# Autodesk Inventor assembly: Main
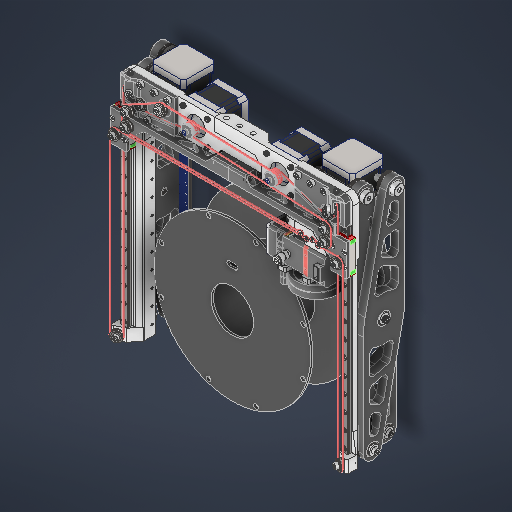
[picture p0: Inventor's stored thumbnail of the model, 512x512]
Saved by Autodesk Inventor 2026.2 (Build 302298000, 298)
## iProperties
Created: 2025-11-20
Part Number: Main
Document SubType Name: Assembly
Designer: gaoet
Author: gaoet
## Documents named in this file (66)
- C:\Users\gaoet\OneDrive\Desktop\Portable3DPrinter\V2\Main.iam
- C:\Users\gaoet\OneDrive\Desktop\Portable3DPrinter\V2\Zeee6S22Ah.ipt
- C:\Users\gaoet\OneDrive\Desktop\Portable3DPrinter\V2\BoundingBox.ipt
- C:\Users\gaoet\OneDrive\Desktop\Portable3DPrinter\V2\BuildVolume.ipt
- C:\Users\gaoet\OneDrive\Desktop\Portable3DPrinter\V2\LaptopScaleModel.ipt
- C:\Users\gaoet\OneDrive\Desktop\Portable3DPrinter\V2\Raspberry PI Zero W\Raspberry PI Zero W.iam
- C:\Users\gaoet\OneDrive\Desktop\Portable3DPrinter\V2\BTT E3 SKR MINI V3.0\BTT E3 SKR MINI V3.0.iam
- C:\Users\gaoet\OneDrive\Desktop\Portable3DPrinter\V2\MGN9-H\MGN9-H\MGN9-H.ipt
- C:\Users\gaoet\OneDrive\Desktop\Portable3DPrinter\V2\ElectronicsBase.ipt
- C:\Users\gaoet\OneDrive\Desktop\Portable3DPrinter\V2\Pololu Stepper with 300mm LeadScrew\Pololu Stepper with 300mm LeadScrew\Pololu Stepper with 300mm LeadScrew.ipt
- C:\Users\gaoet\OneDrive\Desktop\Portable3DPrinter\V2\ScissorArmV2.ipt
- C:\Users\gaoet\OneDrive\Desktop\Portable3DPrinter\V2\7804K117_Stainless Steel Ball Bearing\7804K117_Stainless Steel Ball Bearing\7804K117_Stainless Steel Ball Bearing.ipt
- C:\Users\gaoet\OneDrive\Desktop\Portable3DPrinter\V2\92981A207_Alloy Steel Shoulder Screws\92981A207_Alloy Steel Shoulder Screws\92981A207_Alloy Steel Shoulder Screws.ipt
- C:\Users\gaoet\OneDrive\Desktop\Portable3DPrinter\V2\91415A210_Zinc-Plated Steel Hex Nut\91415A210_Zinc-Plated Steel Hex Nut\91415A210_Zinc-Plated Steel Hex Nut.ipt
- C:\Users\gaoet\OneDrive\Desktop\Portable3DPrinter\V2\CarriagePivotMount.ipt
- C:\Users\gaoet\OneDrive\Desktop\Portable3DPrinter\V2\91290A306_Black-Oxide Alloy Steel Socket Head Screw\91290A306_Black-Oxide Alloy Steel Socket Head Screw\91290A306_Black-Oxide Alloy Steel Socket Head Screw.ipt
- C:\Users\gaoet\OneDrive\Desktop\Portable3DPrinter\V2\PivotWasher.ipt
- C:\Users\gaoet\OneDrive\Desktop\Portable3DPrinter\V2\90591A255_Zinc-Plated Steel Hex Nut\90591A255_Zinc-Plated Steel Hex Nut\90591A255_Zinc-Plated Steel Hex Nut.ipt
- C:\Users\gaoet\OneDrive\Desktop\Portable3DPrinter\V2\ScissorArmV2Inner.ipt
- C:\Users\gaoet\OneDrive\Desktop\Portable3DPrinter\V2\6656K108_Steel Ball Bearing\6656K108_Steel Ball Bearing\6656K108_Steel Ball Bearing.ipt
- C:\Users\gaoet\OneDrive\Desktop\Portable3DPrinter\V2\91290A168_Black-Oxide Alloy Steel Socket Head Screw\91290A168_Black-Oxide Alloy Steel Socket Head Screw\91290A168_Black-Oxide Alloy Steel Socket Head Screw.ipt
- C:\Users\gaoet\OneDrive\Desktop\Portable3DPrinter\V2\ThrustBearing.iam
- C:\Users\gaoet\OneDrive\Desktop\Portable3DPrinter\V2\MGN9-C v2 v0\MGN9-C v2.iam
- C:\Users\gaoet\OneDrive\Desktop\Portable3DPrinter\V2\UpperCarriagePivotMount.ipt
- C:\Users\gaoet\OneDrive\Desktop\Portable3DPrinter\V2\MGN9-H\MGN9-H\MGN9-H_MIR.ipt
- C:\Users\gaoet\OneDrive\Desktop\Portable3DPrinter\V2\91415A210_Zinc-Plated Steel Hex Nut\91415A210_Zinc-Plated Steel Hex Nut\91415A210_Zinc-Plated Steel Hex Nut_MIR.ipt
- C:\Users\gaoet\OneDrive\Desktop\Portable3DPrinter\V2\7804K117_Stainless Steel Ball Bearing\7804K117_Stainless Steel Ball Bearing\7804K117_Stainless Steel Ball Bearing_MIR.ipt
- C:\Users\gaoet\OneDrive\Desktop\Portable3DPrinter\V2\ScissorArmV2_MIR.ipt
- C:\Users\gaoet\OneDrive\Desktop\Portable3DPrinter\V2\92981A207_Alloy Steel Shoulder Screws\92981A207_Alloy Steel Shoulder Screws\92981A207_Alloy Steel Shoulder Screws_MIR.ipt
- C:\Users\gaoet\OneDrive\Desktop\Portable3DPrinter\V2\CarriagePivotMount_MIR.ipt
- C:\Users\gaoet\OneDrive\Desktop\Portable3DPrinter\V2\91290A306_Black-Oxide Alloy Steel Socket Head Screw\91290A306_Black-Oxide Alloy Steel Socket Head Screw\91290A306_Black-Oxide Alloy Steel Socket Head Screw_MIR.ipt
- C:\Users\gaoet\OneDrive\Desktop\Portable3DPrinter\V2\PivotWasher_MIR.ipt
- C:\Users\gaoet\OneDrive\Desktop\Portable3DPrinter\V2\90591A255_Zinc-Plated Steel Hex Nut\90591A255_Zinc-Plated Steel Hex Nut\90591A255_Zinc-Plated Steel Hex Nut_MIR.ipt
- C:\Users\gaoet\OneDrive\Desktop\Portable3DPrinter\V2\ScissorArmV2Inner_MIR.ipt
- C:\Users\gaoet\OneDrive\Desktop\Portable3DPrinter\V2\6656K108_Steel Ball Bearing\6656K108_Steel Ball Bearing\6656K108_Steel Ball Bearing_MIR.ipt
- C:\Users\gaoet\OneDrive\Desktop\Portable3DPrinter\V2\91290A168_Black-Oxide Alloy Steel Socket Head Screw\91290A168_Black-Oxide Alloy Steel Socket Head Screw\91290A168_Black-Oxide Alloy Steel Socket Head Screw_MIR.ipt
- C:\Users\gaoet\OneDrive\Desktop\Portable3DPrinter\V2\ThrustBearing_MIR.iam
- C:\Users\gaoet\OneDrive\Desktop\Portable3DPrinter\V2\MGN9-C v2 v0\MGN9-C v2_MIR.iam
- C:\Users\gaoet\OneDrive\Desktop\Portable3DPrinter\V2\UpperCarriagePivotMount_MIR.ipt
- C:\Users\gaoet\OneDrive\Desktop\Portable3DPrinter\V2\91290A110_Black-Oxide Alloy Steel Socket Head Screw\91290A110_Black-Oxide Alloy Steel Socket Head Screw\91290A110_Black-Oxide Alloy Steel Socket Head Screw_MIR.ipt
- C:\Users\gaoet\OneDrive\Desktop\Portable3DPrinter\V2\GantryRailMount_MIR.ipt
- C:\Users\gaoet\OneDrive\Desktop\Portable3DPrinter\V2\Extruder.iam
- C:\Users\gaoet\OneDrive\Desktop\Portable3DPrinter\V2\MGNRail250mm.ipt
- C:\Users\gaoet\OneDrive\Desktop\Portable3DPrinter\V2\XGantryMount.ipt
- C:\Users\gaoet\OneDrive\Desktop\Portable3DPrinter\V2\BearingU604.ipt
- C:\Users\gaoet\OneDrive\Desktop\Portable3DPrinter\V2\90729A168_Passivated 316 Stainless Steel Hex-Drive Flat Head Screw\90729A168_Passivated 316 Stainless Steel Hex-Drive Flat Head Screw\90729A168_Passivated 316 .ipt
- C:\Users\gaoet\OneDrive\Desktop\Portable3DPrinter\V2\ElevatorPlate.ipt
- C:\Users\gaoet\OneDrive\Desktop\Portable3DPrinter\V2\ElevatorPlate_MIR.ipt
- C:\Users\gaoet\OneDrive\Desktop\Portable3DPrinter\V2\XGantryMount_MIR.ipt
- C:\Users\gaoet\OneDrive\Desktop\Portable3DPrinter\V2\Pulley.ipt
- C:\Users\gaoet\OneDrive\Desktop\Portable3DPrinter\V2\Tensioner.ipt
- C:\Users\gaoet\OneDrive\Desktop\Portable3DPrinter\V2\PSU.ipt
- C:\Users\gaoet\OneDrive\Desktop\Portable3DPrinter\V2\FrontPanel.ipt
- C:\Users\gaoet\OneDrive\Desktop\Portable3DPrinter\V2\BTT Mini 12864 V1.0\BTT Mini 12864 V1.0\BTT Mini 12864 V1.0.ipt
- C:\Users\gaoet\OneDrive\Desktop\Portable3DPrinter\V2\RightTruss.ipt
- C:\Users\gaoet\OneDrive\Desktop\Portable3DPrinter\V2\LeftTruss.ipt
- C:\Users\gaoet\OneDrive\Desktop\Portable3DPrinter\V2\RoutingPlateV2.ipt
- C:\Users\gaoet\OneDrive\Desktop\Portable3DPrinter\V2\RoutingPlateV2Right.ipt
- C:\Users\gaoet\OneDrive\Desktop\Portable3DPrinter\V2\92095A181_NO THREADS_18-8 Stainless Steel Button Head Hex-Drive Screw\92095A181_NO THREADS_18-8 Stainless Steel Button Head Hex-Drive Screw\92095A181_NO THREAD.ipt
- C:\Users\gaoet\OneDrive\Desktop\Portable3DPrinter\V2\MockCable.ipt
- C:\Users\gaoet\OneDrive\Desktop\Portable3DPrinter\V2\MockCable2.ipt
- C:\Users\gaoet\OneDrive\Desktop\Portable3DPrinter\V2\Banana\Banana\Banana.ipt
- C:\Users\gaoet\OneDrive\Desktop\Portable3DPrinter\V2\GantryRailMount.ipt
- C:\Users\gaoet\OneDrive\Desktop\Portable3DPrinter\V2\cardboard spool v1\cardboard spool v1\cardboard spool v1.ipt
- C:\Users\gaoet\OneDrive\Desktop\Portable3DPrinter\Scissor 3D Printer\Nema17x38mm.ipt
- C:\Users\gaoet\OneDrive\Desktop\Portable3DPrinter\Scissor 3D Printer\Pololu Stepper with 300mm LeadScrew\Pololu Stepper with 300mm LeadScrew\Pololu Stepper with 300mm LeadScrew.ipt
## Components (259 placed, 64 different names)
1. Zeee6S22Ah:1
2. BoundingBox:1 — Angle:2, Mate:149, Flush:47
3. BuildVolume:1
4. LaptopScaleModel:1
5. Raspberry PI Zero W:1 [sub-assembly] — Insert:264, Insert:265
6. BTT E3 SKR MINI V3.0:1 [sub-assembly]
7. MGN9-H:2 — Insert:39, Mate:61, Mate:185
8. MGN9-H:3 — Mate:111, Flush:33, Insert:310
9. MGN9-H:6 — Mate:112, Flush:30, Insert:123, Mate:116
10. ElectronicsBase:1 — Mate:149, Flush:47, Mate:156, Flush:49, Insert:203, Insert:206, Insert:210, Insert:214, Insert:215
11. 91415A210_Zinc-Plated Steel Hex Nut:1 — Mate:56
12. 7804K117_Stainless Steel Ball Bearing:2 — Mate:70, Insert:52, Insert:325
13. ScissorArmV2:3 — Insert:35, Angle:2, Mate:73, Insert:63, Insert:64, Insert:71, Insert:74, Insert:78, Angle:4
14. 7804K117_Stainless Steel Ball Bearing:3 — Insert:35, Insert:37
15. 92981A207_Alloy Steel Shoulder Screws:3 — Insert:37, Mate:56
16. CarriagePivotMount:1 — Insert:39, Mate:61, Insert:53, Insert:72
17. 91290A306_Black-Oxide Alloy Steel Socket Head Screw:1 — Mate:70, Insert:51
18. PivotWasher:1 — Insert:51, Insert:52
19. 90591A255_Zinc-Plated Steel Hex Nut:1 — Insert:53
20. ScissorArmV2Inner:1 — Mate:73, Insert:68, Mate:74, Insert:73, Angle:4, Insert:316, Insert:325, Insert:326
21. 7804K117_Stainless Steel Ball Bearing:6 — Insert:63, Insert:66
22. 6656K108_Steel Ball Bearing:1 — Insert:64, Insert:65
23. 6656K108_Steel Ball Bearing:2 — Insert:65
24. PivotWasher:3 — Insert:66, Insert:67
25. 91290A168_Black-Oxide Alloy Steel Socket Head Screw:2 — Insert:67
26. 90591A255_Zinc-Plated Steel Hex Nut:2 — Insert:68, Mate:74
27. ThrustBearing:1 [sub-assembly] — Insert:71
28. ThrustBearing:2 [sub-assembly] — Insert:72, Insert:73
29. MGN9-C v2:1 [sub-assembly] — Mate:80, Insert:308, Flush:51
30. 7804K117_Stainless Steel Ball Bearing:7 — Insert:74, Insert:76
31. PivotWasher:4 — Insert:76, Insert:88
32. ThrustBearing:3 [sub-assembly] — Insert:78, Mate:77, Mate:78
33. UpperCarriagePivotMount:1 — Mate:77, Mate:78, Mate:80, Insert:89, Mate:89, Insert:292, Insert:293, Insert:294, Insert:295, Insert:308
34. 91290A306_Black-Oxide Alloy Steel Socket Head Screw:3 — Insert:88
35. 90591A255_Zinc-Plated Steel Hex Nut:3 — Insert:89, Mate:89
36. MGN9-H_MIR:1 — Mate:94, Insert:93
37. 91415A210_Zinc-Plated Steel Hex Nut_MIR:1 — Mate:93
38. 7804K117_Stainless Steel Ball Bearing_MIR:1 — Mate:95, Insert:94, Insert:324
39. ScissorArmV2_MIR:1 — Insert:90, Angle:6, Mate:96, Insert:98, Insert:99, Insert:104, Insert:107, Insert:109
40. 7804K117_Stainless Steel Ball Bearing_MIR:2 — Insert:90, Insert:91
41. 92981A207_Alloy Steel Shoulder Screws_MIR:1 — Mate:93, Insert:91
42. CarriagePivotMount_MIR:1 — Mate:94, Insert:93, Insert:96, Insert:106
43. 91290A306_Black-Oxide Alloy Steel Socket Head Screw_MIR:1 — Mate:95, Insert:95
44. PivotWasher_MIR:1 — Insert:94, Insert:95
45. 90591A255_Zinc-Plated Steel Hex Nut_MIR:1 — Insert:96
46. ScissorArmV2Inner_MIR:1 — Angle:6, Mate:96, Mate:97, Insert:103, Insert:105, Insert:317, Insert:324, Insert:327, Mate:186
47. 7804K117_Stainless Steel Ball Bearing_MIR:3 — Insert:98, Insert:101
48. 6656K108_Steel Ball Bearing_MIR:1 — Insert:99, Insert:100
49. 6656K108_Steel Ball Bearing_MIR:2 — Insert:100, Mate:186
50. PivotWasher_MIR:2 — Insert:101, Insert:102
51. 91290A168_Black-Oxide Alloy Steel Socket Head Screw_MIR:1 — Insert:102
52. 90591A255_Zinc-Plated Steel Hex Nut_MIR:2 — Mate:97, Insert:103
53. ThrustBearing_MIR:1 [sub-assembly] — Insert:104
54. ThrustBearing_MIR:2 [sub-assembly] — Insert:105, Insert:106
55. MGN9-C v2_MIR:1 [sub-assembly] — Mate:99, Mate:122, Flush:35, Insert:307
56. 7804K117_Stainless Steel Ball Bearing_MIR:4 — Insert:107, Insert:108
57. PivotWasher_MIR:3 — Insert:108, Insert:116
58. ThrustBearing_MIR:3 [sub-assembly] — Insert:109, Mate:100, Mate:101
59. UpperCarriagePivotMount_MIR:1 — Mate:99, Mate:100, Mate:101, Mate:106, Insert:117, Insert:296, Insert:297, Insert:298, Insert:299, Insert:307
60. 91290A306_Black-Oxide Alloy Steel Socket Head Screw_MIR:2 — Insert:116
61. 90591A255_Zinc-Plated Steel Hex Nut_MIR:3 — Mate:106, Insert:117
62. Extruder:1 [sub-assembly] — Insert:310, Insert:311, Insert:312, Insert:313, Insert:314
63. MGNRail250mm:3 — Mate:111, Insert:124, Flush:33, Mate:117, Insert:260
64. MGNRail250mm:4 — Mate:112, Flush:30, Insert:152, Mate:128, Insert:319, Insert:320
65. XGantryMount:1 — Insert:123, Mate:116, Insert:124, Mate:117, Insert:138, Insert:139, Insert:140, Insert:141, Mate:126, Insert:142, Insert:145, Mate:131, Flush:42, Insert:183, Insert:184, Mate:174, Angle:12
66. GantryRailMount_MIR:1 — Insert:132, Insert:133, Insert:134, Insert:135, Insert:153
67. MGNRail250mm:6 — Mate:122, Flush:35, Insert:132, Insert:133, Insert:287
68. MGN9-H:7 — Insert:154, Mate:135
69. MGNRail250mm:7 — Insert:134, Insert:135, Insert:247, Mate:188
70. BearingU604:1 — Insert:147, Insert:321
71. BearingU604:2 — Insert:145, Insert:146
72. BearingU604:3 — Mate:126, Insert:142, Insert:143
73. BearingU604:4 — Insert:156, Insert:158, Mate:178
74. BearingU604:5 — Insert:155, Insert:159
75. BearingU604:6 — Insert:153, Insert:157, Mate:179
76. 90729A168_Passivated 316 :1 — Insert:140
77. 90729A168_Passivated 316 :2 — Insert:141
78. 90729A168_Passivated 316 :3 — Insert:139
79. 90729A168_Passivated 316 :4 — Insert:138
80. 91290A306_Black-Oxide Alloy Steel Socket Head Screw:4 — Insert:143, Mate:175
81. 91290A306_Black-Oxide Alloy Steel Socket Head Screw:5 — Insert:146
82. 91290A306_Black-Oxide Alloy Steel Socket Head Screw:6 — Insert:147
83. 90729A168_Passivated 316 :5 — Insert:312
84. 90729A168_Passivated 316 :6 — Insert:313
85. 90729A168_Passivated 316 :7 — Mate:173, Insert:314
86. 90729A168_Passivated 316 :8 — Insert:311
87. ElevatorPlate:1 — Insert:152, Mate:128, Mate:131, Flush:40, Flush:41, Insert:216, Insert:217, Insert:258, Mate:180, Insert:322, Insert:323, Insert:334, Mate:189
88. ElevatorPlate_MIR:1 — Flush:40, Flush:41, Insert:223, Insert:259, Mate:180, Mate:188, Insert:335, Mate:190
89. XGantryMount_MIR:1 — Insert:154, Mate:135, Flush:42, Insert:155, Insert:156, Insert:160, Insert:161, Insert:162, Insert:163
90. 91290A306_Black-Oxide Alloy Steel Socket Head Screw:7 — Insert:157
91. 91290A306_Black-Oxide Alloy Steel Socket Head Screw:8 — Insert:158
92. 91290A306_Black-Oxide Alloy Steel Socket Head Screw:9 — Insert:159
93. 90729A168_Passivated 316 :9 — Insert:163
94. 90729A168_Passivated 316 :10 — Insert:162
95. 90729A168_Passivated 316 :11 — Insert:161
96. 90729A168_Passivated 316 :12 — Insert:160
97. 92981A207_Alloy Steel Shoulder Screws:4 — Insert:165
98. ThrustBearing:4 [sub-assembly] — Insert:316
99. 7804K117_Stainless Steel Ball Bearing:8 — Insert:165, Insert:326
100. 91415A210_Zinc-Plated Steel Hex Nut:3
101. 92981A207_Alloy Steel Shoulder Screws:5 — Insert:176
102. ThrustBearing:5 [sub-assembly] — Insert:317
103. 7804K117_Stainless Steel Ball Bearing_MIR:5 — Insert:176, Insert:327
104. MGNRail250mm:8 — Mate:185
105. MGNRail250mm:9 — Insert:285
106. BearingU604:10 — Insert:218, Insert:219
107. BearingU604:12 — Insert:187
108. 91290A306_Black-Oxide Alloy Steel Socket Head Screw:20 — Insert:184
109. 91290A306_Black-Oxide Alloy Steel Socket Head Screw:21 — Insert:183
110. Pulley:1 — Mate:192, Flush:55
111. Pulley:2 — Mate:191, Flush:55
112. BearingU604:17 — Insert:229, Insert:231
113. Tensioner:1 — Insert:187, Mate:159, Insert:220, Mate:176, Mate:182
114. PSU:1
115. FrontPanel:2 — Mate:156, Flush:49, Angle:11, Insert:199, Insert:200
116. BTT Mini 12864 V1.0:1 — Angle:11, Insert:199, Insert:200
117. 90729A168_Passivated 316 :15 — Insert:203
118. 90729A168_Passivated 316 :16 — Insert:206
119. 90729A168_Passivated 316 :17 — Insert:210
120. RightTruss:1
121. LeftTruss:1
122. 90729A168_Passivated 316 :19 — Insert:214
123. 90729A168_Passivated 316 :20 — Insert:215
124. RoutingPlateV2:1 — Insert:216, Insert:217, Mate:159, Insert:218, Insert:221, Insert:248, Insert:249, Insert:250, Insert:251, Insert:257, Mate:176, Mate:182
125. 91290A306_Black-Oxide Alloy Steel Socket Head Screw:22 — Insert:219
126. 91290A306_Black-Oxide Alloy Steel Socket Head Screw:23 — Insert:220
127. BearingU604:18 — Insert:221, Insert:222
128. 91290A306_Black-Oxide Alloy Steel Socket Head Screw:24 — Insert:222
129. RoutingPlateV2Right:1 — Insert:223, Insert:225, Mate:164, Insert:228, Insert:229, Insert:252, Insert:253, Insert:254, Insert:255, Insert:256, Mate:177, Mate:183
130. BearingU604:19 — Insert:225, Insert:232
131. BearingU604:21
132. Tensioner:2 — Mate:164, Mate:177, Mate:183
133. 91290A306_Black-Oxide Alloy Steel Socket Head Screw:25
134. BearingU604:22 — Insert:228, Insert:230
135. 91290A306_Black-Oxide Alloy Steel Socket Head Screw:26 — Insert:230
136. 91290A306_Black-Oxide Alloy Steel Socket Head Screw:27 — Insert:231
137. 91290A306_Black-Oxide Alloy Steel Socket Head Screw:28 — Insert:232
138. 91290A306_Black-Oxide Alloy Steel Socket Head Screw:29 — Insert:249
139. 91290A306_Black-Oxide Alloy Steel Socket Head Screw:30 — Insert:251
140. 91290A306_Black-Oxide Alloy Steel Socket Head Screw:31 — Insert:250
141. 91290A306_Black-Oxide Alloy Steel Socket Head Screw:32 — Insert:248
142. 91290A306_Black-Oxide Alloy Steel Socket Head Screw:33 — Insert:255
143. 91290A306_Black-Oxide Alloy Steel Socket Head Screw:34 — Insert:254
144. 91290A306_Black-Oxide Alloy Steel Socket Head Screw:35 — Insert:252
145. 91290A306_Black-Oxide Alloy Steel Socket Head Screw:36 — Insert:253
146. 91290A110_Black-Oxide Alloy Steel Socket Head Screw_MIR:31 — Insert:257
147. 91290A110_Black-Oxide Alloy Steel Socket Head Screw_MIR:32 — Insert:256
148. 91290A110_Black-Oxide Alloy Steel Socket Head Screw_MIR:61 — Insert:264
149. 91290A110_Black-Oxide Alloy Steel Socket Head Screw_MIR:62 — Insert:265
150. 91290A306_Black-Oxide Alloy Steel Socket Head Screw:55
151. 91290A110_Black-Oxide Alloy Steel Socket Head Screw_MIR:115
152. 91290A110_Black-Oxide Alloy Steel Socket Head Screw_MIR:116
153. 91290A110_Black-Oxide Alloy Steel Socket Head Screw_MIR:117
154. 91290A110_Black-Oxide Alloy Steel Socket Head Screw_MIR:118
155. 92095A181_NO THREAD:1 — Insert:295
156. 92095A181_NO THREAD:2 — Insert:294
157. 92095A181_NO THREAD:3 — Insert:293
158. 92095A181_NO THREAD:4 — Insert:292
159. 92095A181_NO THREAD:5 — Insert:296
160. 92095A181_NO THREAD:6 — Insert:297
161. 92095A181_NO THREAD:7 — Insert:298
162. 92095A181_NO THREAD:8 — Insert:299
163. MockCable:1 — Mate:173, Mate:174, Angle:12, Mate:175
164. MockCable2:1 — Mate:178, Mate:179
165. Banana:1
166. GantryRailMount:1 — Insert:319, Insert:320, Insert:321
167. MGNRail250mm:10 — Insert:322, Insert:323, Flush:51
168. cardboard spool v1:1
169. Pololu Stepper with 300mm LeadScrew:2
170. Nema17x38mm:1 — Insert:334, Mate:189, Mate:192
171. Nema17x38mm:2 — Insert:335, Mate:190, Mate:191
172. Pololu Stepper with 300mm LeadScrew:3
173. Pololu Stepper with 300mm LeadScrew:4
174. 91290A110_Black-Oxide Alloy Steel Socket Head Screw_MIR:5 — Insert:247
175. 91290A110_Black-Oxide Alloy Steel Socket Head Screw_MIR:18
176. 91290A110_Black-Oxide Alloy Steel Socket Head Screw_MIR:6
177. 91290A110_Black-Oxide Alloy Steel Socket Head Screw_MIR:19
178. 91290A110_Black-Oxide Alloy Steel Socket Head Screw_MIR:7
179. 91290A110_Black-Oxide Alloy Steel Socket Head Screw_MIR:20
180. 91290A110_Black-Oxide Alloy Steel Socket Head Screw_MIR:8
181. 91290A110_Black-Oxide Alloy Steel Socket Head Screw_MIR:21
182. 91290A110_Black-Oxide Alloy Steel Socket Head Screw_MIR:9
183. 91290A110_Black-Oxide Alloy Steel Socket Head Screw_MIR:22
184. 91290A110_Black-Oxide Alloy Steel Socket Head Screw_MIR:10
185. 91290A110_Black-Oxide Alloy Steel Socket Head Screw_MIR:23
186. 91290A110_Black-Oxide Alloy Steel Socket Head Screw_MIR:11
187. 91290A110_Black-Oxide Alloy Steel Socket Head Screw_MIR:24
188. 91290A110_Black-Oxide Alloy Steel Socket Head Screw_MIR:12
189. 91290A110_Black-Oxide Alloy Steel Socket Head Screw_MIR:25
190. 91290A110_Black-Oxide Alloy Steel Socket Head Screw_MIR:13
191. 91290A110_Black-Oxide Alloy Steel Socket Head Screw_MIR:26
192. 91290A110_Black-Oxide Alloy Steel Socket Head Screw_MIR:14
193. 91290A110_Black-Oxide Alloy Steel Socket Head Screw_MIR:27
194. 91290A110_Black-Oxide Alloy Steel Socket Head Screw_MIR:15
195. 91290A110_Black-Oxide Alloy Steel Socket Head Screw_MIR:28
196. 91290A110_Black-Oxide Alloy Steel Socket Head Screw_MIR:16
197. 91290A110_Black-Oxide Alloy Steel Socket Head Screw_MIR:29
198. 91290A110_Black-Oxide Alloy Steel Socket Head Screw_MIR:17
199. 91290A110_Black-Oxide Alloy Steel Socket Head Screw_MIR:30
200. 91290A110_Black-Oxide Alloy Steel Socket Head Screw_MIR:41 — Insert:260
201. 91290A110_Black-Oxide Alloy Steel Socket Head Screw_MIR:42
202. 91290A110_Black-Oxide Alloy Steel Socket Head Screw_MIR:43
203. 91290A110_Black-Oxide Alloy Steel Socket Head Screw_MIR:44
204. 91290A110_Black-Oxide Alloy Steel Socket Head Screw_MIR:45
205. 91290A110_Black-Oxide Alloy Steel Socket Head Screw_MIR:46
206. 91290A110_Black-Oxide Alloy Steel Socket Head Screw_MIR:47
207. 91290A110_Black-Oxide Alloy Steel Socket Head Screw_MIR:48
208. 91290A110_Black-Oxide Alloy Steel Socket Head Screw_MIR:49
209. 91290A110_Black-Oxide Alloy Steel Socket Head Screw_MIR:50
210. 91290A110_Black-Oxide Alloy Steel Socket Head Screw_MIR:51
211. 91290A110_Black-Oxide Alloy Steel Socket Head Screw_MIR:52
212. 91290A110_Black-Oxide Alloy Steel Socket Head Screw_MIR:53
213. 91290A110_Black-Oxide Alloy Steel Socket Head Screw_MIR:63 — Insert:285
214. 91290A110_Black-Oxide Alloy Steel Socket Head Screw_MIR:64
215. 91290A110_Black-Oxide Alloy Steel Socket Head Screw_MIR:65
216. 91290A110_Black-Oxide Alloy Steel Socket Head Screw_MIR:66
217. 91290A110_Black-Oxide Alloy Steel Socket Head Screw_MIR:67
218. 91290A110_Black-Oxide Alloy Steel Socket Head Screw_MIR:68
219. 91290A110_Black-Oxide Alloy Steel Socket Head Screw_MIR:69
220. 91290A110_Black-Oxide Alloy Steel Socket Head Screw_MIR:70
221. 91290A110_Black-Oxide Alloy Steel Socket Head Screw_MIR:71
222. 91290A110_Black-Oxide Alloy Steel Socket Head Screw_MIR:72
223. 91290A110_Black-Oxide Alloy Steel Socket Head Screw_MIR:73
224. 91290A110_Black-Oxide Alloy Steel Socket Head Screw_MIR:74
225. 91290A110_Black-Oxide Alloy Steel Socket Head Screw_MIR:75
226. 91290A110_Black-Oxide Alloy Steel Socket Head Screw_MIR:76
227. 91290A110_Black-Oxide Alloy Steel Socket Head Screw_MIR:77
228. 91290A110_Black-Oxide Alloy Steel Socket Head Screw_MIR:78
229. 91290A110_Black-Oxide Alloy Steel Socket Head Screw_MIR:79
230. 91290A110_Black-Oxide Alloy Steel Socket Head Screw_MIR:80
231. 91290A110_Black-Oxide Alloy Steel Socket Head Screw_MIR:81
232. 91290A110_Black-Oxide Alloy Steel Socket Head Screw_MIR:82
233. 91290A110_Black-Oxide Alloy Steel Socket Head Screw_MIR:83
234. 91290A110_Black-Oxide Alloy Steel Socket Head Screw_MIR:84
235. 91290A110_Black-Oxide Alloy Steel Socket Head Screw_MIR:85
236. 91290A110_Black-Oxide Alloy Steel Socket Head Screw_MIR:86
237. 91290A110_Black-Oxide Alloy Steel Socket Head Screw_MIR:87
238. 91290A110_Black-Oxide Alloy Steel Socket Head Screw_MIR:88
239. 91290A110_Black-Oxide Alloy Steel Socket Head Screw_MIR:102 — Insert:287
240. 91290A110_Black-Oxide Alloy Steel Socket Head Screw_MIR:103
241. 91290A110_Black-Oxide Alloy Steel Socket Head Screw_MIR:104
242. 91290A110_Black-Oxide Alloy Steel Socket Head Screw_MIR:105
243. 91290A110_Black-Oxide Alloy Steel Socket Head Screw_MIR:106
244. 91290A110_Black-Oxide Alloy Steel Socket Head Screw_MIR:107
245. 91290A110_Black-Oxide Alloy Steel Socket Head Screw_MIR:108
246. 91290A110_Black-Oxide Alloy Steel Socket Head Screw_MIR:109
247. 91290A110_Black-Oxide Alloy Steel Socket Head Screw_MIR:110
248. 91290A110_Black-Oxide Alloy Steel Socket Head Screw_MIR:111
249. 91290A110_Black-Oxide Alloy Steel Socket Head Screw_MIR:112
250. 91290A110_Black-Oxide Alloy Steel Socket Head Screw_MIR:113
251. 91290A110_Black-Oxide Alloy Steel Socket Head Screw_MIR:114
252. 91290A110_Black-Oxide Alloy Steel Socket Head Screw_MIR:33 — Insert:258
253. 91290A110_Black-Oxide Alloy Steel Socket Head Screw_MIR:130
254. 91290A110_Black-Oxide Alloy Steel Socket Head Screw_MIR:131
255. 91290A110_Black-Oxide Alloy Steel Socket Head Screw_MIR:132
256. 91290A110_Black-Oxide Alloy Steel Socket Head Screw_MIR:37 — Insert:259
257. 91290A110_Black-Oxide Alloy Steel Socket Head Screw_MIR:133
258. 91290A110_Black-Oxide Alloy Steel Socket Head Screw_MIR:134
259. 91290A110_Black-Oxide Alloy Steel Socket Head Screw_MIR:135
## Component patterns: (26 elements, first: 91290A110_Black-Oxide Alloy Steel Socket Head Screw_MIR:5), (13 elements, first: 91290A110_Black-Oxide Alloy Steel Socket Head Screw_MIR:41), (26 elements, first: 91290A110_Black-Oxide Alloy Steel Socket Head Screw_MIR:63), (13 elements, first: 91290A110_Black-Oxide Alloy Steel Socket Head Screw_MIR:102), (4 elements, first: 91290A110_Black-Oxide Alloy Steel Socket Head Screw_MIR:33), (4 elements, first: 91290A110_Black-Oxide Alloy Steel Socket Head Screw_MIR:37)
## Relationships (206: Insert 141, Mate 49, Flush 11, Angle 5)
- Insert:35: ScissorArmV2:3 ↔ 7804K117_Stainless Steel Ball Bearing:3
- Insert:37: 7804K117_Stainless Steel Ball Bearing:3 ↔ 92981A207_Alloy Steel Shoulder Screws:3
- Mate:56: 91415A210_Zinc-Plated Steel Hex Nut:1 ↔ 92981A207_Alloy Steel Shoulder Screws:3
- Angle:2 (186 deg): BoundingBox:1 ↔ ScissorArmV2:3
- Insert:39: MGN9-H:2 ↔ CarriagePivotMount:1
- Mate:61: MGN9-H:2 ↔ CarriagePivotMount:1
- Mate:70: 7804K117_Stainless Steel Ball Bearing:2 ↔ 91290A306_Black-Oxide Alloy Steel Socket Head Screw:1
- Insert:51: 91290A306_Black-Oxide Alloy Steel Socket Head Screw:1 ↔ PivotWasher:1
- Insert:52: 7804K117_Stainless Steel Ball Bearing:2 ↔ PivotWasher:1
- Insert:53: CarriagePivotMount:1 ↔ 90591A255_Zinc-Plated Steel Hex Nut:1
- Mate:73: ScissorArmV2:3 ↔ ScissorArmV2Inner:1
- Insert:63: ScissorArmV2:3 ↔ 7804K117_Stainless Steel Ball Bearing:6
- Insert:64: ScissorArmV2:3 ↔ 6656K108_Steel Ball Bearing:1
- Insert:65: 6656K108_Steel Ball Bearing:1 ↔ 6656K108_Steel Ball Bearing:2
- Insert:66: 7804K117_Stainless Steel Ball Bearing:6 ↔ PivotWasher:3
- Insert:67: PivotWasher:3 ↔ 91290A168_Black-Oxide Alloy Steel Socket Head Screw:2
- Insert:68: ScissorArmV2Inner:1 ↔ 90591A255_Zinc-Plated Steel Hex Nut:2
- Mate:74: ScissorArmV2Inner:1 ↔ 90591A255_Zinc-Plated Steel Hex Nut:2
- Insert:71: ScissorArmV2:3 ↔ ThrustBearing:1
- Insert:72: CarriagePivotMount:1 ↔ ThrustBearing:2
- Insert:73: ScissorArmV2Inner:1 ↔ ThrustBearing:2
- Insert:74: ScissorArmV2:3 ↔ 7804K117_Stainless Steel Ball Bearing:7
- Insert:76: 7804K117_Stainless Steel Ball Bearing:7 ↔ PivotWasher:4
- Insert:78: ScissorArmV2:3 ↔ ThrustBearing:3
- Mate:77: ThrustBearing:3 ↔ UpperCarriagePivotMount:1
- Mate:78: ThrustBearing:3 ↔ UpperCarriagePivotMount:1
- Angle:4 (0 deg): ScissorArmV2:3 ↔ ScissorArmV2Inner:1
- Mate:80: MGN9-C v2:1 ↔ UpperCarriagePivotMount:1
- Insert:88: PivotWasher:4 ↔ 91290A306_Black-Oxide Alloy Steel Socket Head Screw:3
- Insert:89: UpperCarriagePivotMount:1 ↔ 90591A255_Zinc-Plated Steel Hex Nut:3
- Mate:89: UpperCarriagePivotMount:1 ↔ 90591A255_Zinc-Plated Steel Hex Nut:3
- Insert:90: ScissorArmV2_MIR:1 ↔ 7804K117_Stainless Steel Ball Bearing_MIR:2
- Mate:93: 91415A210_Zinc-Plated Steel Hex Nut_MIR:1 ↔ 92981A207_Alloy Steel Shoulder Screws_MIR:1
- Insert:91: 7804K117_Stainless Steel Ball Bearing_MIR:2 ↔ 92981A207_Alloy Steel Shoulder Screws_MIR:1
- Mate:94: MGN9-H_MIR:1 ↔ CarriagePivotMount_MIR:1
- Insert:93: MGN9-H_MIR:1 ↔ CarriagePivotMount_MIR:1
- Mate:95: 7804K117_Stainless Steel Ball Bearing_MIR:1 ↔ 91290A306_Black-Oxide Alloy Steel Socket Head Screw_MIR:1
- Insert:94: 7804K117_Stainless Steel Ball Bearing_MIR:1 ↔ PivotWasher_MIR:1
- Insert:95: 91290A306_Black-Oxide Alloy Steel Socket Head Screw_MIR:1 ↔ PivotWasher_MIR:1
- Insert:96: CarriagePivotMount_MIR:1 ↔ 90591A255_Zinc-Plated Steel Hex Nut_MIR:1
- Angle:6 (0 deg): ScissorArmV2_MIR:1 ↔ ScissorArmV2Inner_MIR:1
- Mate:96: ScissorArmV2_MIR:1 ↔ ScissorArmV2Inner_MIR:1
- Insert:98: ScissorArmV2_MIR:1 ↔ 7804K117_Stainless Steel Ball Bearing_MIR:3
- Insert:99: ScissorArmV2_MIR:1 ↔ 6656K108_Steel Ball Bearing_MIR:1
- Insert:100: 6656K108_Steel Ball Bearing_MIR:1 ↔ 6656K108_Steel Ball Bearing_MIR:2
- Insert:101: 7804K117_Stainless Steel Ball Bearing_MIR:3 ↔ PivotWasher_MIR:2
- Insert:102: PivotWasher_MIR:2 ↔ 91290A168_Black-Oxide Alloy Steel Socket Head Screw_MIR:1
- Mate:97: ScissorArmV2Inner_MIR:1 ↔ 90591A255_Zinc-Plated Steel Hex Nut_MIR:2
- Insert:103: ScissorArmV2Inner_MIR:1 ↔ 90591A255_Zinc-Plated Steel Hex Nut_MIR:2
- Insert:104: ScissorArmV2_MIR:1 ↔ ThrustBearing_MIR:1
- Insert:105: ScissorArmV2Inner_MIR:1 ↔ ThrustBearing_MIR:2
- Insert:106: CarriagePivotMount_MIR:1 ↔ ThrustBearing_MIR:2
- Insert:107: ScissorArmV2_MIR:1 ↔ 7804K117_Stainless Steel Ball Bearing_MIR:4
- Insert:108: 7804K117_Stainless Steel Ball Bearing_MIR:4 ↔ PivotWasher_MIR:3
- Insert:109: ScissorArmV2_MIR:1 ↔ ThrustBearing_MIR:3
- Mate:99: MGN9-C v2_MIR:1 ↔ UpperCarriagePivotMount_MIR:1
- Mate:100: ThrustBearing_MIR:3 ↔ UpperCarriagePivotMount_MIR:1
- Mate:101: ThrustBearing_MIR:3 ↔ UpperCarriagePivotMount_MIR:1
- Insert:116: PivotWasher_MIR:3 ↔ 91290A306_Black-Oxide Alloy Steel Socket Head Screw_MIR:2
- Mate:106: UpperCarriagePivotMount_MIR:1 ↔ 90591A255_Zinc-Plated Steel Hex Nut_MIR:3
- Insert:117: UpperCarriagePivotMount_MIR:1 ↔ 90591A255_Zinc-Plated Steel Hex Nut_MIR:3
- Mate:111: MGN9-H:3 ↔ MGNRail250mm:3
- Mate:112: MGN9-H:6 ↔ MGNRail250mm:4
- Flush:30 (5.5 mm): MGN9-H:6 ↔ MGNRail250mm:4
- Insert:123: MGN9-H:6 ↔ XGantryMount:1
- Mate:116: MGN9-H:6 ↔ XGantryMount:1
- Insert:124: MGNRail250mm:3 ↔ XGantryMount:1
- Flush:33 (-5.5 mm): MGN9-H:3 ↔ MGNRail250mm:3
- Mate:117: MGNRail250mm:3 ↔ XGantryMount:1
- Mate:122: MGN9-C v2_MIR:1 ↔ MGNRail250mm:6
- Flush:35 (5.5 mm): MGN9-C v2_MIR:1 ↔ MGNRail250mm:6
- Insert:132: GantryRailMount_MIR:1 ↔ MGNRail250mm:6
- Insert:133: GantryRailMount_MIR:1 ↔ MGNRail250mm:6
- [Mate]: MGN9-H:7 ↔ MGNRail250mm:7
- [Flush] (5.5 mm): MGN9-H:7 ↔ MGNRail250mm:7
- Insert:134: GantryRailMount_MIR:1 ↔ MGNRail250mm:7
- Insert:135: GantryRailMount_MIR:1 ↔ MGNRail250mm:7
- Insert:138: XGantryMount:1 ↔ 90729A168_Passivated 316 :4
- Insert:139: XGantryMount:1 ↔ 90729A168_Passivated 316 :3
- Insert:140: XGantryMount:1 ↔ 90729A168_Passivated 316 :1
- Insert:141: XGantryMount:1 ↔ 90729A168_Passivated 316 :2
- Mate:126: XGantryMount:1 ↔ BearingU604:3
- Insert:142: XGantryMount:1 ↔ BearingU604:3
- Insert:143: BearingU604:3 ↔ 91290A306_Black-Oxide Alloy Steel Socket Head Screw:4
- Insert:145: XGantryMount:1 ↔ BearingU604:2
- Insert:146: BearingU604:2 ↔ 91290A306_Black-Oxide Alloy Steel Socket Head Screw:5
- Insert:147: BearingU604:1 ↔ 91290A306_Black-Oxide Alloy Steel Socket Head Screw:6
- Insert:152: MGNRail250mm:4 ↔ ElevatorPlate:1
- Mate:128: MGNRail250mm:4 ↔ ElevatorPlate:1
- Mate:131: XGantryMount:1 ↔ ElevatorPlate:1
- Flush:40: ElevatorPlate:1 ↔ ElevatorPlate_MIR:1
- Flush:41: ElevatorPlate:1 ↔ ElevatorPlate_MIR:1
- Insert:153: GantryRailMount_MIR:1 ↔ BearingU604:6
- Insert:154: MGN9-H:7 ↔ XGantryMount_MIR:1
- Mate:135: MGN9-H:7 ↔ XGantryMount_MIR:1
- Flush:42: XGantryMount:1 ↔ XGantryMount_MIR:1
- Insert:155: BearingU604:5 ↔ XGantryMount_MIR:1
- Insert:156: BearingU604:4 ↔ XGantryMount_MIR:1
- Insert:157: BearingU604:6 ↔ 91290A306_Black-Oxide Alloy Steel Socket Head Screw:7
- Insert:158: BearingU604:4 ↔ 91290A306_Black-Oxide Alloy Steel Socket Head Screw:8
- Insert:159: BearingU604:5 ↔ 91290A306_Black-Oxide Alloy Steel Socket Head Screw:9
- Insert:160: XGantryMount_MIR:1 ↔ 90729A168_Passivated 316 :12
- Insert:161: XGantryMount_MIR:1 ↔ 90729A168_Passivated 316 :11
- Insert:162: XGantryMount_MIR:1 ↔ 90729A168_Passivated 316 :10
- Insert:163: XGantryMount_MIR:1 ↔ 90729A168_Passivated 316 :9
- Insert:165: 92981A207_Alloy Steel Shoulder Screws:4 ↔ 7804K117_Stainless Steel Ball Bearing:8
- Insert:176: 92981A207_Alloy Steel Shoulder Screws:5 ↔ 7804K117_Stainless Steel Ball Bearing_MIR:5
- Insert:183: XGantryMount:1 ↔ 91290A306_Black-Oxide Alloy Steel Socket Head Screw:21
- Insert:184: XGantryMount:1 ↔ 91290A306_Black-Oxide Alloy Steel Socket Head Screw:20
- Insert:187: BearingU604:12 ↔ Tensioner:1
- Mate:149: BoundingBox:1 ↔ ElectronicsBase:1
- Flush:47: BoundingBox:1 ↔ ElectronicsBase:1
- Mate:156: ElectronicsBase:1 ↔ FrontPanel:2
- Flush:49: ElectronicsBase:1 ↔ FrontPanel:2
- Angle:11 (0 deg): FrontPanel:2 ↔ BTT Mini 12864 V1.0:1
- Insert:199: FrontPanel:2 ↔ BTT Mini 12864 V1.0:1
- Insert:200: FrontPanel:2 ↔ BTT Mini 12864 V1.0:1
- Insert:203: ElectronicsBase:1 ↔ 90729A168_Passivated 316 :15
- Insert:206: ElectronicsBase:1 ↔ 90729A168_Passivated 316 :16
- Insert:210: ElectronicsBase:1 ↔ 90729A168_Passivated 316 :17
- Insert:214: ElectronicsBase:1 ↔ 90729A168_Passivated 316 :19
- Insert:215: ElectronicsBase:1 ↔ 90729A168_Passivated 316 :20
- Insert:216: ElevatorPlate:1 ↔ RoutingPlateV2:1
- Insert:217: ElevatorPlate:1 ↔ RoutingPlateV2:1
- Mate:159 (0.1 mm): Tensioner:1 ↔ RoutingPlateV2:1
- Insert:218: BearingU604:10 ↔ RoutingPlateV2:1
- Insert:219: BearingU604:10 ↔ 91290A306_Black-Oxide Alloy Steel Socket Head Screw:22
- Insert:220: Tensioner:1 ↔ 91290A306_Black-Oxide Alloy Steel Socket Head Screw:23
- Insert:221: RoutingPlateV2:1 ↔ BearingU604:18
- Insert:222: BearingU604:18 ↔ 91290A306_Black-Oxide Alloy Steel Socket Head Screw:24
- Insert:223: ElevatorPlate_MIR:1 ↔ RoutingPlateV2Right:1
- Insert:225: RoutingPlateV2Right:1 ↔ BearingU604:19
- [Insert]: BearingU604:21 ↔ Tensioner:2
- [Insert]: Tensioner:2 ↔ 91290A306_Black-Oxide Alloy Steel Socket Head Screw:25
- Mate:164 (0.1 mm): RoutingPlateV2Right:1 ↔ Tensioner:2
- Insert:228: RoutingPlateV2Right:1 ↔ BearingU604:22
- Insert:229: BearingU604:17 ↔ RoutingPlateV2Right:1
- Insert:230: BearingU604:22 ↔ 91290A306_Black-Oxide Alloy Steel Socket Head Screw:26
- Insert:231: BearingU604:17 ↔ 91290A306_Black-Oxide Alloy Steel Socket Head Screw:27
- Insert:232: BearingU604:19 ↔ 91290A306_Black-Oxide Alloy Steel Socket Head Screw:28
- Insert:247: MGNRail250mm:7 ↔ 91290A110_Black-Oxide Alloy Steel Socket Head Screw_MIR:5
- Insert:248: RoutingPlateV2:1 ↔ 91290A306_Black-Oxide Alloy Steel Socket Head Screw:32
- Insert:249: RoutingPlateV2:1 ↔ 91290A306_Black-Oxide Alloy Steel Socket Head Screw:29
- Insert:250: RoutingPlateV2:1 ↔ 91290A306_Black-Oxide Alloy Steel Socket Head Screw:31
- Insert:251: RoutingPlateV2:1 ↔ 91290A306_Black-Oxide Alloy Steel Socket Head Screw:30
- Insert:252: RoutingPlateV2Right:1 ↔ 91290A306_Black-Oxide Alloy Steel Socket Head Screw:35
- Insert:253: RoutingPlateV2Right:1 ↔ 91290A306_Black-Oxide Alloy Steel Socket Head Screw:36
- Insert:254: RoutingPlateV2Right:1 ↔ 91290A306_Black-Oxide Alloy Steel Socket Head Screw:34
- Insert:255: RoutingPlateV2Right:1 ↔ 91290A306_Black-Oxide Alloy Steel Socket Head Screw:33
- Insert:256: RoutingPlateV2Right:1 ↔ 91290A110_Black-Oxide Alloy Steel Socket Head Screw_MIR:32
- Insert:257: RoutingPlateV2:1 ↔ 91290A110_Black-Oxide Alloy Steel Socket Head Screw_MIR:31
- Insert:258: ElevatorPlate:1 ↔ 91290A110_Black-Oxide Alloy Steel Socket Head Screw_MIR:33
- Insert:259: ElevatorPlate_MIR:1 ↔ 91290A110_Black-Oxide Alloy Steel Socket Head Screw_MIR:37
- Insert:260: MGNRail250mm:3 ↔ 91290A110_Black-Oxide Alloy Steel Socket Head Screw_MIR:41
- Insert:264: Raspberry PI Zero W:1 ↔ 91290A110_Black-Oxide Alloy Steel Socket Head Screw_MIR:61
- Insert:265: Raspberry PI Zero W:1 ↔ 91290A110_Black-Oxide Alloy Steel Socket Head Screw_MIR:62
- Insert:285: MGNRail250mm:9 ↔ 91290A110_Black-Oxide Alloy Steel Socket Head Screw_MIR:63
- Insert:287: MGNRail250mm:6 ↔ 91290A110_Black-Oxide Alloy Steel Socket Head Screw_MIR:102
- Insert:292: UpperCarriagePivotMount:1 ↔ 92095A181_NO THREAD:4
- Insert:293: UpperCarriagePivotMount:1 ↔ 92095A181_NO THREAD:3
- Insert:294: UpperCarriagePivotMount:1 ↔ 92095A181_NO THREAD:2
- Insert:295: UpperCarriagePivotMount:1 ↔ 92095A181_NO THREAD:1
- Insert:296: UpperCarriagePivotMount_MIR:1 ↔ 92095A181_NO THREAD:5
- Insert:297: UpperCarriagePivotMount_MIR:1 ↔ 92095A181_NO THREAD:6
- Insert:298: UpperCarriagePivotMount_MIR:1 ↔ 92095A181_NO THREAD:7
- Insert:299: UpperCarriagePivotMount_MIR:1 ↔ 92095A181_NO THREAD:8
- Mate:173: 90729A168_Passivated 316 :7 ↔ MockCable:1
- Mate:174 (2.5 mm): XGantryMount:1 ↔ MockCable:1
- Angle:12 (180 deg): XGantryMount:1 ↔ MockCable:1
- Mate:175: 91290A306_Black-Oxide Alloy Steel Socket Head Screw:4 ↔ MockCable:1
- Mate:176: Tensioner:1 ↔ RoutingPlateV2:1
- Mate:177: RoutingPlateV2Right:1 ↔ Tensioner:2
- Mate:178: BearingU604:4 ↔ MockCable2:1
- Mate:179: BearingU604:6 ↔ MockCable2:1
- Mate:180: ElevatorPlate:1 ↔ ElevatorPlate_MIR:1
- Insert:307: MGN9-C v2_MIR:1 ↔ UpperCarriagePivotMount_MIR:1
- Insert:308: MGN9-C v2:1 ↔ UpperCarriagePivotMount:1
- Insert:310: MGN9-H:3 ↔ Extruder:1
- Insert:311 (-2 mm): Extruder:1 ↔ 90729A168_Passivated 316 :8
- Insert:312 (-2 mm): Extruder:1 ↔ 90729A168_Passivated 316 :5
- Insert:313 (-2 mm): Extruder:1 ↔ 90729A168_Passivated 316 :6
- Insert:314 (-2 mm): Extruder:1 ↔ 90729A168_Passivated 316 :7
- Insert:316: ScissorArmV2Inner:1 ↔ ThrustBearing:4
- Insert:317: ScissorArmV2Inner_MIR:1 ↔ ThrustBearing:5
- Mate:182 (0.16 mm): Tensioner:1 ↔ RoutingPlateV2:1
- Mate:183 (0.16 mm): RoutingPlateV2Right:1 ↔ Tensioner:2
- Insert:319: MGNRail250mm:4 ↔ GantryRailMount:1
- Insert:320: MGNRail250mm:4 ↔ GantryRailMount:1
- Insert:321: BearingU604:1 ↔ GantryRailMount:1
- Insert:322: ElevatorPlate:1 ↔ MGNRail250mm:10
- Insert:323: ElevatorPlate:1 ↔ MGNRail250mm:10
- Flush:51 (-5.5 mm): MGN9-C v2:1 ↔ MGNRail250mm:10
- Insert:324: 7804K117_Stainless Steel Ball Bearing_MIR:1 ↔ ScissorArmV2Inner_MIR:1
- Insert:325: 7804K117_Stainless Steel Ball Bearing:2 ↔ ScissorArmV2Inner:1
- Insert:326: ScissorArmV2Inner:1 ↔ 7804K117_Stainless Steel Ball Bearing:8
- Insert:327: ScissorArmV2Inner_MIR:1 ↔ 7804K117_Stainless Steel Ball Bearing_MIR:5
- Mate:185: MGN9-H:2 ↔ MGNRail250mm:8
- Mate:186: ScissorArmV2Inner_MIR:1 ↔ 6656K108_Steel Ball Bearing_MIR:2
- Mate:188: MGNRail250mm:7 ↔ ElevatorPlate_MIR:1
- Insert:334: ElevatorPlate:1 ↔ Nema17x38mm:1
- Mate:189: ElevatorPlate:1 ↔ Nema17x38mm:1
- Insert:335: ElevatorPlate_MIR:1 ↔ Nema17x38mm:2
- Mate:190: ElevatorPlate_MIR:1 ↔ Nema17x38mm:2
- Mate:191: Pulley:2 ↔ Nema17x38mm:2
- Mate:192: Pulley:1 ↔ Nema17x38mm:1
- Flush:55: Pulley:1 ↔ Pulley:2
## Named parameters: d361_d326 = 0 mm, d362_d327 = 5.5 mm, d552_d463 = 0 mm, d553_d540 = 0 mm
